# Autodesk Inventor assembly: mixer
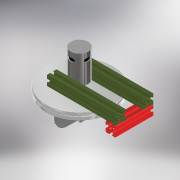
[picture p0: Inventor's stored thumbnail of the model, 180x180]
Saved by Autodesk Inventor 2020 (Build 240168000, 168)
## iProperties
Created: 2020-06-18
Part Number: mixer
Document SubType Name: Assembly
Designer: pc-konvi
Author: pc-konvi
## Documents named in this file (8)
- C:\Users\pc-konvi\Documents\Lobola\open_source_scrabble\lobola - rapid prototype\mixer.iam
- C:\Users\pc-konvi\Documents\Lobola\open_source_scrabble\lobola - rapid prototype\dc_motor.ipt
- C:\Users\pc-konvi\Documents\Lobola\open_source_scrabble\lobola - rapid prototype\Pot_Lid.ipt
- C:\Users\pc-konvi\Documents\Lobola\open_source_scrabble\lobola - rapid prototype\lid_holder.ipt
- C:\Users\pc-konvi\Documents\Lobola\open_source_scrabble\lobola - rapid prototype\screw_platform.ipt
- C:\Users\pc-konvi\Documents\Lobola\open_source_scrabble\lobola - rapid prototype\blade.ipt
- C:\Users\pc-konvi\Documents\Lobola\open_source_scrabble\lobola - rapid prototype\blade_rod.ipt
- C:\Users\pc-konvi\Documents\Lobola\open_source_scrabble\lobola - rapid prototype\mixer_coupler.ipt
## Components (9 placed, 8 different names)
1. dc_motor:1 — Mate:1, Mate:2, Mate:3, Mate:4, Mate:5, Mate:6, Flush:2, Flush:3, Flush:4, Mate:15
2. Pot_Lid:1 — Mate:4, Mate:5, Mate:6, Mate:14
3. lid_holder_left — Mate:7, Flush:1, Mate:8, Flush:2
4. lid_holder_right — Mate:7, Flush:1, Mate:8, Flush:3, Flush:4, Flush:10, Mate:9, Flush:11
5. screw_platform:1 — Flush:10, Mate:9, Flush:11
6. blade_rod:1 — Mate:10, Mate:11, Flush:12, Flush:13
7. mixer_coupler:1 — Mate:10, Mate:11, Mate:14, Mate:15
8. blade:2 — Mate:16, Flush:12, Flush:13, Flush:14, Mate:17, Mate:18
9. blade:3 — Flush:14, Mate:17, Mate:18
## Relationships (25: Mate 16, Flush 9)
- Mate:1: dc_motor:1
- Mate:2: dc_motor:1
- Mate:3: dc_motor:1
- Mate:4: dc_motor:1 ↔ Pot_Lid:1
- Mate:5: dc_motor:1 ↔ Pot_Lid:1
- Mate:6 (5 mm): dc_motor:1 ↔ Pot_Lid:1
- Mate:7: lid_holder_left ↔ lid_holder_right
- Flush:1: lid_holder_left ↔ lid_holder_right
- Mate:8 (52 mm): lid_holder_left ↔ lid_holder_right
- Flush:2 (65 mm): dc_motor:1 ↔ lid_holder_left
- Flush:3 (-40.9 mm): dc_motor:1 ↔ lid_holder_right
- Flush:4 (-26 mm): dc_motor:1 ↔ lid_holder_right
- Flush:10: lid_holder_right ↔ screw_platform:1
- Mate:9: lid_holder_right ↔ screw_platform:1
- Flush:11: lid_holder_right ↔ screw_platform:1
- Mate:10: blade_rod:1 ↔ mixer_coupler:1
- Mate:11: blade_rod:1 ↔ mixer_coupler:1
- Mate:14: Pot_Lid:1 ↔ mixer_coupler:1
- Mate:15 (-10 mm): dc_motor:1 ↔ mixer_coupler:1
- Mate:16 (4 mm): blade:2
- Flush:12: blade_rod:1 ↔ blade:2
- Flush:13 (-4 mm): blade_rod:1 ↔ blade:2
- Flush:14: blade:2 ↔ blade:3
- Mate:17 (8 mm): blade:2 ↔ blade:3
- Mate:18 (-8 mm): blade:2 ↔ blade:3
